# Autodesk Inventor assembly: Bumper Frame
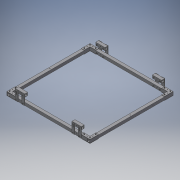
[picture p0: Inventor's stored thumbnail of the model, 180x180]
Saved by Autodesk Inventor 2018 (Build 220112000, 112)
## iProperties
Created: 2019-01-21
Part Number: Bumper Frame
Document SubType Name: Assembly
Designer: maste
Author: maste
## Documents named in this file (8)
- C:\Users\s-2512711\Desktop\Github\2019CAD\Drivebase but Calvin is a mad man\Bumper Frame.iam
- C:\Users\s-2512711\Desktop\Github\2019CAD\Drivebase but Calvin is a mad man\1x1 29in.ipt
- C:\Users\s-2512711\Desktop\Github\2019CAD\Drivebase but Calvin is a mad man\1x1 27in.ipt
- C:\Users\s-2512711\Desktop\Github\2019CAD\Drivebase but Calvin is a mad man\L gusset 2.ipt
- C:\Users\s-2512711\Desktop\Github\2019CAD\Drivebase but Calvin is a mad man\Slot Bumper attachment.ipt
- C:\Users\s-2512711\Desktop\Github\2019CAD\Drivebase but Calvin is a mad man\1x1 Bumper Attachment.ipt
- C:\Users\s-2512711\Desktop\Github\2019CAD\Drivebase but Calvin is a mad man\92196A251_18-8 STAINLESS STEEL SOCKET HEAD CAP SCREW.ipt
- C:\Users\s-2512711\Desktop\Github\2019CAD\Drivebase but Calvin is a mad man\91831A011_TYPE 18-8 STAINLESS STL NYLON-INSERT LOCKNUT.ipt
## Components (80 placed, 7 different names)
1. 1x1 29in:1 — Mate:1, Flush:1, Flush:2, Mate:10, Mate:12, Mate:13, Mate:14, Mate:16, Mate:18, Mate:19, Mate:21
2. 1x1 29in:2 — Mate:2, Flush:3, Flush:4, Mate:3, Flush:5, Flush:6, Mate:4, Mate:5, Mate:7, Mate:9, Mate:24, Mate:26
3. 1x1 27in:1 — Mate:1, Flush:1, Flush:2, Mate:2, Flush:3, Flush:4, Mate:6, Mate:8, Mate:11, Mate:15, Mate:36, Mate:37, Mate:38, Mate:39, Flush:11, Flush:12, Mate:40, Mate:41, Mate:42, Mate:43, Flush:13, Flush:14, Mate:96, Mate:97, Mate:98, Mate:99
4. 1x1 27in:2 — Mate:3, Flush:5, Flush:6, Mate:17, Mate:20, Mate:22, Mate:23, Mate:25, Mate:27, Mate:28, Mate:29, Flush:7, Mate:30, Mate:31, Flush:8, Mate:32, Mate:33, Mate:34, Flush:9, Mate:35, Flush:10, Mate:92, Mate:93, Mate:94, Mate:95
5. L gusset 2:1 — Mate:16, Mate:17, Mate:18, Mate:114, Mate:115, Mate:116
6. L gusset 2:2 — Mate:19, Mate:20, Mate:21, Mate:64, Mate:65, Mate:66, Mate:67, Mate:68, Mate:69
7. L gusset 2:3 — Mate:25, Mate:26, Mate:27, Mate:58, Mate:59, Mate:60, Mate:61, Mate:62, Mate:63
8. L gusset 2:4 — Mate:22, Mate:23, Mate:24, Mate:117, Mate:118, Mate:119
9. L gusset 2:5 — Mate:7, Mate:8, Mate:9, Mate:111, Mate:112, Mate:113
10. L gusset 2:6 — Mate:4, Mate:5, Mate:6, Mate:52, Mate:53, Mate:54, Mate:55, Mate:56, Mate:57
11. L gusset 2:7 — Mate:10, Mate:11, Mate:12, Mate:108, Mate:109, Mate:110
12. L gusset 2:8 — Mate:13, Mate:14, Mate:15, Mate:70, Mate:71, Mate:72, Mate:73, Mate:74, Mate:75
13. Slot Bumper attachment:1 — Mate:32, Mate:35, Flush:10, Mate:44, Mate:45, Flush:15, Mate:87, Mate:91, Mate:149, Mate:150
14. Slot Bumper attachment:2 — Mate:40, Mate:43, Flush:13, Mate:78, Mate:82, Mate:157, Mate:158
15. Slot Bumper attachment:3 — Mate:30, Mate:31, Flush:8, Mate:46, Mate:47, Flush:16, Mate:85, Mate:89, Mate:140, Mate:143
16. Slot Bumper attachment:4 — Mate:28, Mate:29, Flush:7, Mate:84, Mate:88, Mate:141, Mate:142
17. Slot Bumper attachment:5 — Mate:36, Mate:39, Flush:12, Mate:76, Mate:80, Mate:132, Mate:135
18. Slot Bumper attachment:6 — Mate:37, Mate:38, Flush:11, Mate:50, Mate:51, Flush:18, Mate:77, Mate:81, Mate:133, Mate:134
19. Slot Bumper attachment:7 — Mate:33, Mate:34, Flush:9, Mate:86, Mate:90, Mate:148, Mate:151
20. Slot Bumper attachment:8 — Mate:41, Mate:42, Flush:14, Mate:48, Mate:49, Flush:17, Mate:79, Mate:83, Mate:156, Mate:159
21. 1x1 Bumper Attachment:1 — Mate:46, Mate:47, Flush:16, Mate:144, Mate:145
22. 1x1 Bumper Attachment:2 — Mate:50, Mate:51, Flush:18, Mate:136, Mate:137
23. 1x1 Bumper Attachment:3 — Mate:48, Mate:49, Flush:17, Mate:160, Mate:161
24. 1x1 Bumper Attachment:4 — Mate:44, Mate:45, Flush:15, Mate:152, Mate:153
25. 92196A251_18-8 STAINLESS STEEL SOCKET HEAD CAP SCREW:1 — Mate:65, Mate:68, Mate:124
26. 92196A251_18-8 STAINLESS STEEL SOCKET HEAD CAP SCREW:2 — Mate:64, Mate:67, Mate:125
27. 92196A251_18-8 STAINLESS STEEL SOCKET HEAD CAP SCREW:3 — Mate:66, Mate:69, Mate:123
28. 92196A251_18-8 STAINLESS STEEL SOCKET HEAD CAP SCREW:4 — Mate:70, Mate:73, Mate:126
29. 92196A251_18-8 STAINLESS STEEL SOCKET HEAD CAP SCREW:5 — Mate:71, Mate:74, Mate:127
30. 92196A251_18-8 STAINLESS STEEL SOCKET HEAD CAP SCREW:6 — Mate:72, Mate:75, Mate:128
31. 92196A251_18-8 STAINLESS STEEL SOCKET HEAD CAP SCREW:7 — Mate:52, Mate:57, Mate:129
32. 92196A251_18-8 STAINLESS STEEL SOCKET HEAD CAP SCREW:8 — Mate:53, Mate:56, Mate:130
33. 92196A251_18-8 STAINLESS STEEL SOCKET HEAD CAP SCREW:9 — Mate:54, Mate:55, Mate:131
34. 92196A251_18-8 STAINLESS STEEL SOCKET HEAD CAP SCREW:10 — Mate:58, Mate:62, Mate:120
35. 92196A251_18-8 STAINLESS STEEL SOCKET HEAD CAP SCREW:11 — Mate:59, Mate:61, Mate:121
36. 92196A251_18-8 STAINLESS STEEL SOCKET HEAD CAP SCREW:12 — Mate:60, Mate:63, Mate:122
37. 92196A251_18-8 STAINLESS STEEL SOCKET HEAD CAP SCREW:13 — Mate:78, Mate:82, Mate:100
38. 92196A251_18-8 STAINLESS STEEL SOCKET HEAD CAP SCREW:14 — Mate:79, Mate:83, Mate:101
39. 92196A251_18-8 STAINLESS STEEL SOCKET HEAD CAP SCREW:15 — Mate:77, Mate:81, Mate:102
40. 92196A251_18-8 STAINLESS STEEL SOCKET HEAD CAP SCREW:16 — Mate:76, Mate:80, Mate:103
41. 92196A251_18-8 STAINLESS STEEL SOCKET HEAD CAP SCREW:17 — Mate:84, Mate:88, Mate:105
42. 92196A251_18-8 STAINLESS STEEL SOCKET HEAD CAP SCREW:18 — Mate:85, Mate:89, Mate:104
43. 92196A251_18-8 STAINLESS STEEL SOCKET HEAD CAP SCREW:19 — Mate:86, Mate:90, Mate:106
44. 92196A251_18-8 STAINLESS STEEL SOCKET HEAD CAP SCREW:20 — Mate:87, Mate:91, Mate:107
45. 91831A011_TYPE 18-8 STAINLESS STL NYLON-INSERT LOCKNUT:1 — Mate:110, Mate:128
46. 91831A011_TYPE 18-8 STAINLESS STL NYLON-INSERT LOCKNUT:2 — Mate:108, Mate:127
47. 91831A011_TYPE 18-8 STAINLESS STL NYLON-INSERT LOCKNUT:3 — Mate:109, Mate:126
48. 91831A011_TYPE 18-8 STAINLESS STL NYLON-INSERT LOCKNUT:4 — Mate:114, Mate:125
49. 91831A011_TYPE 18-8 STAINLESS STL NYLON-INSERT LOCKNUT:5 — Mate:115, Mate:124
50. 91831A011_TYPE 18-8 STAINLESS STL NYLON-INSERT LOCKNUT:6 — Mate:116, Mate:123
51. 91831A011_TYPE 18-8 STAINLESS STL NYLON-INSERT LOCKNUT:7 — Mate:117, Mate:122
52. 91831A011_TYPE 18-8 STAINLESS STL NYLON-INSERT LOCKNUT:8 — Mate:118, Mate:121
53. 91831A011_TYPE 18-8 STAINLESS STL NYLON-INSERT LOCKNUT:9 — Mate:119, Mate:120
54. 91831A011_TYPE 18-8 STAINLESS STL NYLON-INSERT LOCKNUT:10 — Mate:113, Mate:131
55. 91831A011_TYPE 18-8 STAINLESS STL NYLON-INSERT LOCKNUT:11 — Mate:112, Mate:130
56. 91831A011_TYPE 18-8 STAINLESS STL NYLON-INSERT LOCKNUT:12 — Mate:111, Mate:129
57. 91831A011_TYPE 18-8 STAINLESS STL NYLON-INSERT LOCKNUT:13 — Mate:98, Mate:100
58. 91831A011_TYPE 18-8 STAINLESS STL NYLON-INSERT LOCKNUT:14 — Mate:99, Mate:101
59. 91831A011_TYPE 18-8 STAINLESS STL NYLON-INSERT LOCKNUT:15 — Mate:97, Mate:102
60. 91831A011_TYPE 18-8 STAINLESS STL NYLON-INSERT LOCKNUT:16 — Mate:96, Mate:103
61. 91831A011_TYPE 18-8 STAINLESS STL NYLON-INSERT LOCKNUT:17 — Mate:95, Mate:105
62. 91831A011_TYPE 18-8 STAINLESS STL NYLON-INSERT LOCKNUT:18 — Mate:94, Mate:104
63. 91831A011_TYPE 18-8 STAINLESS STL NYLON-INSERT LOCKNUT:19 — Mate:92, Mate:106
64. 91831A011_TYPE 18-8 STAINLESS STL NYLON-INSERT LOCKNUT:20 — Mate:93, Mate:107
65. 92196A251_18-8 STAINLESS STEEL SOCKET HEAD CAP SCREW:21 — Mate:132, Mate:135, Mate:139
66. 92196A251_18-8 STAINLESS STEEL SOCKET HEAD CAP SCREW:22 — Mate:133, Mate:134, Mate:138
67. 92196A251_18-8 STAINLESS STEEL SOCKET HEAD CAP SCREW:23 — Mate:157, Mate:158, Mate:162
68. 92196A251_18-8 STAINLESS STEEL SOCKET HEAD CAP SCREW:24 — Mate:156, Mate:159, Mate:163
69. 92196A251_18-8 STAINLESS STEEL SOCKET HEAD CAP SCREW:25 — Mate:148, Mate:151, Mate:155
70. 92196A251_18-8 STAINLESS STEEL SOCKET HEAD CAP SCREW:26 — Mate:149, Mate:150, Mate:154
71. 92196A251_18-8 STAINLESS STEEL SOCKET HEAD CAP SCREW:27 — Mate:140, Mate:143, Mate:147
72. 92196A251_18-8 STAINLESS STEEL SOCKET HEAD CAP SCREW:28 — Mate:141, Mate:142, Mate:146
73. 91831A011_TYPE 18-8 STAINLESS STL NYLON-INSERT LOCKNUT:21 — Mate:145, Mate:146
74. 91831A011_TYPE 18-8 STAINLESS STL NYLON-INSERT LOCKNUT:22 — Mate:144, Mate:147
75. 91831A011_TYPE 18-8 STAINLESS STL NYLON-INSERT LOCKNUT:23 — Mate:152, Mate:155
76. 91831A011_TYPE 18-8 STAINLESS STL NYLON-INSERT LOCKNUT:24 — Mate:153, Mate:154
77. 91831A011_TYPE 18-8 STAINLESS STL NYLON-INSERT LOCKNUT:25 — Mate:160, Mate:163
78. 91831A011_TYPE 18-8 STAINLESS STL NYLON-INSERT LOCKNUT:26 — Mate:161, Mate:162
79. 91831A011_TYPE 18-8 STAINLESS STL NYLON-INSERT LOCKNUT:27 — Mate:137, Mate:138
80. 91831A011_TYPE 18-8 STAINLESS STL NYLON-INSERT LOCKNUT:28 — Mate:136, Mate:139
## Relationships (181: Mate 163, Flush 18)
- Mate:1: 1x1 29in:1 ↔ 1x1 27in:1
- Flush:1: 1x1 29in:1 ↔ 1x1 27in:1
- Flush:2: 1x1 29in:1 ↔ 1x1 27in:1
- Mate:2: 1x1 29in:2 ↔ 1x1 27in:1
- Flush:3: 1x1 29in:2 ↔ 1x1 27in:1
- Flush:4: 1x1 29in:2 ↔ 1x1 27in:1
- Mate:3: 1x1 29in:2 ↔ 1x1 27in:2
- Flush:5: 1x1 29in:2 ↔ 1x1 27in:2
- Flush:6: 1x1 29in:2 ↔ 1x1 27in:2
- Mate:4: 1x1 29in:2 ↔ L gusset 2:6
- Mate:5: 1x1 29in:2 ↔ L gusset 2:6
- Mate:6: 1x1 27in:1 ↔ L gusset 2:6
- Mate:7: 1x1 29in:2 ↔ L gusset 2:5
- Mate:8: 1x1 27in:1 ↔ L gusset 2:5
- Mate:9: 1x1 29in:2 ↔ L gusset 2:5
- Mate:10: 1x1 29in:1 ↔ L gusset 2:7
- Mate:11: 1x1 27in:1 ↔ L gusset 2:7
- Mate:12: 1x1 29in:1 ↔ L gusset 2:7
- Mate:13: 1x1 29in:1 ↔ L gusset 2:8
- Mate:14: 1x1 29in:1 ↔ L gusset 2:8
- Mate:15: 1x1 27in:1 ↔ L gusset 2:8
- Mate:16: 1x1 29in:1 ↔ L gusset 2:1
- Mate:17: 1x1 27in:2 ↔ L gusset 2:1
- Mate:18: 1x1 29in:1 ↔ L gusset 2:1
- Mate:19: 1x1 29in:1 ↔ L gusset 2:2
- Mate:20: 1x1 27in:2 ↔ L gusset 2:2
- Mate:21: 1x1 29in:1 ↔ L gusset 2:2
- Mate:22: 1x1 27in:2 ↔ L gusset 2:4
- Mate:23: 1x1 27in:2 ↔ L gusset 2:4
- Mate:24: 1x1 29in:2 ↔ L gusset 2:4
- Mate:25: 1x1 27in:2 ↔ L gusset 2:3
- Mate:26: 1x1 29in:2 ↔ L gusset 2:3
- Mate:27: 1x1 27in:2 ↔ L gusset 2:3
- Mate:28: 1x1 27in:2 ↔ Slot Bumper attachment:4
- Mate:29: 1x1 27in:2 ↔ Slot Bumper attachment:4
- Flush:7: 1x1 27in:2 ↔ Slot Bumper attachment:4
- Mate:30: 1x1 27in:2 ↔ Slot Bumper attachment:3
- Mate:31: 1x1 27in:2 ↔ Slot Bumper attachment:3
- Flush:8: 1x1 27in:2 ↔ Slot Bumper attachment:3
- Mate:32: 1x1 27in:2 ↔ Slot Bumper attachment:1
- Mate:33: 1x1 27in:2 ↔ Slot Bumper attachment:7
- Mate:34: 1x1 27in:2 ↔ Slot Bumper attachment:7
- Flush:9: 1x1 27in:2 ↔ Slot Bumper attachment:7
- Mate:35: 1x1 27in:2 ↔ Slot Bumper attachment:1
- Flush:10: 1x1 27in:2 ↔ Slot Bumper attachment:1
- Mate:36: 1x1 27in:1 ↔ Slot Bumper attachment:5
- Mate:37: 1x1 27in:1 ↔ Slot Bumper attachment:6
- Mate:38: 1x1 27in:1 ↔ Slot Bumper attachment:6
- Mate:39: 1x1 27in:1 ↔ Slot Bumper attachment:5
- Flush:11: 1x1 27in:1 ↔ Slot Bumper attachment:6
- Flush:12: 1x1 27in:1 ↔ Slot Bumper attachment:5
- Mate:40: 1x1 27in:1 ↔ Slot Bumper attachment:2
- Mate:41: 1x1 27in:1 ↔ Slot Bumper attachment:8
- Mate:42: 1x1 27in:1 ↔ Slot Bumper attachment:8
- Mate:43: 1x1 27in:1 ↔ Slot Bumper attachment:2
- Flush:13: 1x1 27in:1 ↔ Slot Bumper attachment:2
- Flush:14: 1x1 27in:1 ↔ Slot Bumper attachment:8
- Mate:44: Slot Bumper attachment:1 ↔ 1x1 Bumper Attachment:4
- Mate:45: Slot Bumper attachment:1 ↔ 1x1 Bumper Attachment:4
- Flush:15: Slot Bumper attachment:1 ↔ 1x1 Bumper Attachment:4
- Mate:46: Slot Bumper attachment:3 ↔ 1x1 Bumper Attachment:1
- Mate:47: Slot Bumper attachment:3 ↔ 1x1 Bumper Attachment:1
- Flush:16: Slot Bumper attachment:3 ↔ 1x1 Bumper Attachment:1
- Mate:48: Slot Bumper attachment:8 ↔ 1x1 Bumper Attachment:3
- Mate:49: Slot Bumper attachment:8 ↔ 1x1 Bumper Attachment:3
- Flush:17: Slot Bumper attachment:8 ↔ 1x1 Bumper Attachment:3
- Mate:50: Slot Bumper attachment:6 ↔ 1x1 Bumper Attachment:2
- Mate:51: Slot Bumper attachment:6 ↔ 1x1 Bumper Attachment:2
- Flush:18: Slot Bumper attachment:6 ↔ 1x1 Bumper Attachment:2
- Mate:52: L gusset 2:6 ↔ 92196A251_18-8 STAINLESS STEEL SOCKET HEAD CAP SCREW:7
- Mate:53: L gusset 2:6 ↔ 92196A251_18-8 STAINLESS STEEL SOCKET HEAD CAP SCREW:8
- Mate:54: L gusset 2:6 ↔ 92196A251_18-8 STAINLESS STEEL SOCKET HEAD CAP SCREW:9
- Mate:55: L gusset 2:6 ↔ 92196A251_18-8 STAINLESS STEEL SOCKET HEAD CAP SCREW:9
- Mate:56: L gusset 2:6 ↔ 92196A251_18-8 STAINLESS STEEL SOCKET HEAD CAP SCREW:8
- Mate:57: L gusset 2:6 ↔ 92196A251_18-8 STAINLESS STEEL SOCKET HEAD CAP SCREW:7
- Mate:58: L gusset 2:3 ↔ 92196A251_18-8 STAINLESS STEEL SOCKET HEAD CAP SCREW:10
- Mate:59: L gusset 2:3 ↔ 92196A251_18-8 STAINLESS STEEL SOCKET HEAD CAP SCREW:11
- Mate:60: L gusset 2:3 ↔ 92196A251_18-8 STAINLESS STEEL SOCKET HEAD CAP SCREW:12
- Mate:61: L gusset 2:3 ↔ 92196A251_18-8 STAINLESS STEEL SOCKET HEAD CAP SCREW:11
- Mate:62: L gusset 2:3 ↔ 92196A251_18-8 STAINLESS STEEL SOCKET HEAD CAP SCREW:10
- Mate:63: L gusset 2:3 ↔ 92196A251_18-8 STAINLESS STEEL SOCKET HEAD CAP SCREW:12
- Mate:64: L gusset 2:2 ↔ 92196A251_18-8 STAINLESS STEEL SOCKET HEAD CAP SCREW:2
- Mate:65: L gusset 2:2 ↔ 92196A251_18-8 STAINLESS STEEL SOCKET HEAD CAP SCREW:1
- Mate:66: L gusset 2:2 ↔ 92196A251_18-8 STAINLESS STEEL SOCKET HEAD CAP SCREW:3
- Mate:67: L gusset 2:2 ↔ 92196A251_18-8 STAINLESS STEEL SOCKET HEAD CAP SCREW:2
- Mate:68: L gusset 2:2 ↔ 92196A251_18-8 STAINLESS STEEL SOCKET HEAD CAP SCREW:1
- Mate:69: L gusset 2:2 ↔ 92196A251_18-8 STAINLESS STEEL SOCKET HEAD CAP SCREW:3
- Mate:70: L gusset 2:8 ↔ 92196A251_18-8 STAINLESS STEEL SOCKET HEAD CAP SCREW:4
- Mate:71: L gusset 2:8 ↔ 92196A251_18-8 STAINLESS STEEL SOCKET HEAD CAP SCREW:5
- Mate:72: L gusset 2:8 ↔ 92196A251_18-8 STAINLESS STEEL SOCKET HEAD CAP SCREW:6
- Mate:73: L gusset 2:8 ↔ 92196A251_18-8 STAINLESS STEEL SOCKET HEAD CAP SCREW:4
- Mate:74: L gusset 2:8 ↔ 92196A251_18-8 STAINLESS STEEL SOCKET HEAD CAP SCREW:5
- Mate:75: L gusset 2:8 ↔ 92196A251_18-8 STAINLESS STEEL SOCKET HEAD CAP SCREW:6
- Mate:76: Slot Bumper attachment:5 ↔ 92196A251_18-8 STAINLESS STEEL SOCKET HEAD CAP SCREW:16
- Mate:77: Slot Bumper attachment:6 ↔ 92196A251_18-8 STAINLESS STEEL SOCKET HEAD CAP SCREW:15
- Mate:78: Slot Bumper attachment:2 ↔ 92196A251_18-8 STAINLESS STEEL SOCKET HEAD CAP SCREW:13
- Mate:79: Slot Bumper attachment:8 ↔ 92196A251_18-8 STAINLESS STEEL SOCKET HEAD CAP SCREW:14
- Mate:80: Slot Bumper attachment:5 ↔ 92196A251_18-8 STAINLESS STEEL SOCKET HEAD CAP SCREW:16
- Mate:81: Slot Bumper attachment:6 ↔ 92196A251_18-8 STAINLESS STEEL SOCKET HEAD CAP SCREW:15
- Mate:82: Slot Bumper attachment:2 ↔ 92196A251_18-8 STAINLESS STEEL SOCKET HEAD CAP SCREW:13
- Mate:83: Slot Bumper attachment:8 ↔ 92196A251_18-8 STAINLESS STEEL SOCKET HEAD CAP SCREW:14
- Mate:84: Slot Bumper attachment:4 ↔ 92196A251_18-8 STAINLESS STEEL SOCKET HEAD CAP SCREW:17
- Mate:85: Slot Bumper attachment:3 ↔ 92196A251_18-8 STAINLESS STEEL SOCKET HEAD CAP SCREW:18
- Mate:86: Slot Bumper attachment:7 ↔ 92196A251_18-8 STAINLESS STEEL SOCKET HEAD CAP SCREW:19
- Mate:87: Slot Bumper attachment:1 ↔ 92196A251_18-8 STAINLESS STEEL SOCKET HEAD CAP SCREW:20
- Mate:88: Slot Bumper attachment:4 ↔ 92196A251_18-8 STAINLESS STEEL SOCKET HEAD CAP SCREW:17
- Mate:89: Slot Bumper attachment:3 ↔ 92196A251_18-8 STAINLESS STEEL SOCKET HEAD CAP SCREW:18
- Mate:90: Slot Bumper attachment:7 ↔ 92196A251_18-8 STAINLESS STEEL SOCKET HEAD CAP SCREW:19
- Mate:91: Slot Bumper attachment:1 ↔ 92196A251_18-8 STAINLESS STEEL SOCKET HEAD CAP SCREW:20
- Mate:92: 1x1 27in:2 ↔ 91831A011_TYPE 18-8 STAINLESS STL NYLON-INSERT LOCKNUT:19
- Mate:93: 1x1 27in:2 ↔ 91831A011_TYPE 18-8 STAINLESS STL NYLON-INSERT LOCKNUT:20
- Mate:94: 1x1 27in:2 ↔ 91831A011_TYPE 18-8 STAINLESS STL NYLON-INSERT LOCKNUT:18
- Mate:95: 1x1 27in:2 ↔ 91831A011_TYPE 18-8 STAINLESS STL NYLON-INSERT LOCKNUT:17
- Mate:96: 1x1 27in:1 ↔ 91831A011_TYPE 18-8 STAINLESS STL NYLON-INSERT LOCKNUT:16
- Mate:97: 1x1 27in:1 ↔ 91831A011_TYPE 18-8 STAINLESS STL NYLON-INSERT LOCKNUT:15
- Mate:98: 1x1 27in:1 ↔ 91831A011_TYPE 18-8 STAINLESS STL NYLON-INSERT LOCKNUT:13
- Mate:99: 1x1 27in:1 ↔ 91831A011_TYPE 18-8 STAINLESS STL NYLON-INSERT LOCKNUT:14
- Mate:100: 92196A251_18-8 STAINLESS STEEL SOCKET HEAD CAP SCREW:13 ↔ 91831A011_TYPE 18-8 STAINLESS STL NYLON-INSERT LOCKNUT:13
- Mate:101: 92196A251_18-8 STAINLESS STEEL SOCKET HEAD CAP SCREW:14 ↔ 91831A011_TYPE 18-8 STAINLESS STL NYLON-INSERT LOCKNUT:14
- Mate:102: 92196A251_18-8 STAINLESS STEEL SOCKET HEAD CAP SCREW:15 ↔ 91831A011_TYPE 18-8 STAINLESS STL NYLON-INSERT LOCKNUT:15
- Mate:103: 92196A251_18-8 STAINLESS STEEL SOCKET HEAD CAP SCREW:16 ↔ 91831A011_TYPE 18-8 STAINLESS STL NYLON-INSERT LOCKNUT:16
- Mate:104: 92196A251_18-8 STAINLESS STEEL SOCKET HEAD CAP SCREW:18 ↔ 91831A011_TYPE 18-8 STAINLESS STL NYLON-INSERT LOCKNUT:18
- Mate:105: 92196A251_18-8 STAINLESS STEEL SOCKET HEAD CAP SCREW:17 ↔ 91831A011_TYPE 18-8 STAINLESS STL NYLON-INSERT LOCKNUT:17
- Mate:106: 92196A251_18-8 STAINLESS STEEL SOCKET HEAD CAP SCREW:19 ↔ 91831A011_TYPE 18-8 STAINLESS STL NYLON-INSERT LOCKNUT:19
- Mate:107: 92196A251_18-8 STAINLESS STEEL SOCKET HEAD CAP SCREW:20 ↔ 91831A011_TYPE 18-8 STAINLESS STL NYLON-INSERT LOCKNUT:20
- Mate:108: L gusset 2:7 ↔ 91831A011_TYPE 18-8 STAINLESS STL NYLON-INSERT LOCKNUT:2
- Mate:109: L gusset 2:7 ↔ 91831A011_TYPE 18-8 STAINLESS STL NYLON-INSERT LOCKNUT:3
- Mate:110: L gusset 2:7 ↔ 91831A011_TYPE 18-8 STAINLESS STL NYLON-INSERT LOCKNUT:1
- Mate:111: L gusset 2:5 ↔ 91831A011_TYPE 18-8 STAINLESS STL NYLON-INSERT LOCKNUT:12
- Mate:112: L gusset 2:5 ↔ 91831A011_TYPE 18-8 STAINLESS STL NYLON-INSERT LOCKNUT:11
- Mate:113: L gusset 2:5 ↔ 91831A011_TYPE 18-8 STAINLESS STL NYLON-INSERT LOCKNUT:10
- Mate:114: L gusset 2:1 ↔ 91831A011_TYPE 18-8 STAINLESS STL NYLON-INSERT LOCKNUT:4
- Mate:115: L gusset 2:1 ↔ 91831A011_TYPE 18-8 STAINLESS STL NYLON-INSERT LOCKNUT:5
- Mate:116: L gusset 2:1 ↔ 91831A011_TYPE 18-8 STAINLESS STL NYLON-INSERT LOCKNUT:6
- Mate:117: L gusset 2:4 ↔ 91831A011_TYPE 18-8 STAINLESS STL NYLON-INSERT LOCKNUT:7
- Mate:118: L gusset 2:4 ↔ 91831A011_TYPE 18-8 STAINLESS STL NYLON-INSERT LOCKNUT:8
- Mate:119: L gusset 2:4 ↔ 91831A011_TYPE 18-8 STAINLESS STL NYLON-INSERT LOCKNUT:9
- Mate:120: 92196A251_18-8 STAINLESS STEEL SOCKET HEAD CAP SCREW:10 ↔ 91831A011_TYPE 18-8 STAINLESS STL NYLON-INSERT LOCKNUT:9
- Mate:121: 92196A251_18-8 STAINLESS STEEL SOCKET HEAD CAP SCREW:11 ↔ 91831A011_TYPE 18-8 STAINLESS STL NYLON-INSERT LOCKNUT:8
- Mate:122: 92196A251_18-8 STAINLESS STEEL SOCKET HEAD CAP SCREW:12 ↔ 91831A011_TYPE 18-8 STAINLESS STL NYLON-INSERT LOCKNUT:7
- Mate:123: 92196A251_18-8 STAINLESS STEEL SOCKET HEAD CAP SCREW:3 ↔ 91831A011_TYPE 18-8 STAINLESS STL NYLON-INSERT LOCKNUT:6
- Mate:124: 92196A251_18-8 STAINLESS STEEL SOCKET HEAD CAP SCREW:1 ↔ 91831A011_TYPE 18-8 STAINLESS STL NYLON-INSERT LOCKNUT:5
- Mate:125: 92196A251_18-8 STAINLESS STEEL SOCKET HEAD CAP SCREW:2 ↔ 91831A011_TYPE 18-8 STAINLESS STL NYLON-INSERT LOCKNUT:4
- Mate:126: 92196A251_18-8 STAINLESS STEEL SOCKET HEAD CAP SCREW:4 ↔ 91831A011_TYPE 18-8 STAINLESS STL NYLON-INSERT LOCKNUT:3
- Mate:127: 92196A251_18-8 STAINLESS STEEL SOCKET HEAD CAP SCREW:5 ↔ 91831A011_TYPE 18-8 STAINLESS STL NYLON-INSERT LOCKNUT:2
- Mate:128: 92196A251_18-8 STAINLESS STEEL SOCKET HEAD CAP SCREW:6 ↔ 91831A011_TYPE 18-8 STAINLESS STL NYLON-INSERT LOCKNUT:1
- Mate:129: 92196A251_18-8 STAINLESS STEEL SOCKET HEAD CAP SCREW:7 ↔ 91831A011_TYPE 18-8 STAINLESS STL NYLON-INSERT LOCKNUT:12
- Mate:130: 92196A251_18-8 STAINLESS STEEL SOCKET HEAD CAP SCREW:8 ↔ 91831A011_TYPE 18-8 STAINLESS STL NYLON-INSERT LOCKNUT:11
- Mate:131: 92196A251_18-8 STAINLESS STEEL SOCKET HEAD CAP SCREW:9 ↔ 91831A011_TYPE 18-8 STAINLESS STL NYLON-INSERT LOCKNUT:10
- Mate:132: Slot Bumper attachment:5 ↔ 92196A251_18-8 STAINLESS STEEL SOCKET HEAD CAP SCREW:21
- Mate:133: Slot Bumper attachment:6 ↔ 92196A251_18-8 STAINLESS STEEL SOCKET HEAD CAP SCREW:22
- Mate:134: Slot Bumper attachment:6 ↔ 92196A251_18-8 STAINLESS STEEL SOCKET HEAD CAP SCREW:22
- Mate:135: Slot Bumper attachment:5 ↔ 92196A251_18-8 STAINLESS STEEL SOCKET HEAD CAP SCREW:21
- Mate:136: 1x1 Bumper Attachment:2 ↔ 91831A011_TYPE 18-8 STAINLESS STL NYLON-INSERT LOCKNUT:28
- Mate:137: 1x1 Bumper Attachment:2 ↔ 91831A011_TYPE 18-8 STAINLESS STL NYLON-INSERT LOCKNUT:27
- Mate:138: 92196A251_18-8 STAINLESS STEEL SOCKET HEAD CAP SCREW:22 ↔ 91831A011_TYPE 18-8 STAINLESS STL NYLON-INSERT LOCKNUT:27
- Mate:139: 92196A251_18-8 STAINLESS STEEL SOCKET HEAD CAP SCREW:21 ↔ 91831A011_TYPE 18-8 STAINLESS STL NYLON-INSERT LOCKNUT:28
- Mate:140: Slot Bumper attachment:3 ↔ 92196A251_18-8 STAINLESS STEEL SOCKET HEAD CAP SCREW:27
- Mate:141: Slot Bumper attachment:4 ↔ 92196A251_18-8 STAINLESS STEEL SOCKET HEAD CAP SCREW:28
- Mate:142: Slot Bumper attachment:4 ↔ 92196A251_18-8 STAINLESS STEEL SOCKET HEAD CAP SCREW:28
- Mate:143: Slot Bumper attachment:3 ↔ 92196A251_18-8 STAINLESS STEEL SOCKET HEAD CAP SCREW:27
- Mate:144: 1x1 Bumper Attachment:1 ↔ 91831A011_TYPE 18-8 STAINLESS STL NYLON-INSERT LOCKNUT:22
- Mate:145: 1x1 Bumper Attachment:1 ↔ 91831A011_TYPE 18-8 STAINLESS STL NYLON-INSERT LOCKNUT:21
- Mate:146: 92196A251_18-8 STAINLESS STEEL SOCKET HEAD CAP SCREW:28 ↔ 91831A011_TYPE 18-8 STAINLESS STL NYLON-INSERT LOCKNUT:21
- Mate:147: 92196A251_18-8 STAINLESS STEEL SOCKET HEAD CAP SCREW:27 ↔ 91831A011_TYPE 18-8 STAINLESS STL NYLON-INSERT LOCKNUT:22
- Mate:148: Slot Bumper attachment:7 ↔ 92196A251_18-8 STAINLESS STEEL SOCKET HEAD CAP SCREW:25
- Mate:149: Slot Bumper attachment:1 ↔ 92196A251_18-8 STAINLESS STEEL SOCKET HEAD CAP SCREW:26
- Mate:150: Slot Bumper attachment:1 ↔ 92196A251_18-8 STAINLESS STEEL SOCKET HEAD CAP SCREW:26
- Mate:151: Slot Bumper attachment:7 ↔ 92196A251_18-8 STAINLESS STEEL SOCKET HEAD CAP SCREW:25
- Mate:152: 1x1 Bumper Attachment:4 ↔ 91831A011_TYPE 18-8 STAINLESS STL NYLON-INSERT LOCKNUT:23
- Mate:153: 1x1 Bumper Attachment:4 ↔ 91831A011_TYPE 18-8 STAINLESS STL NYLON-INSERT LOCKNUT:24
- Mate:154: 92196A251_18-8 STAINLESS STEEL SOCKET HEAD CAP SCREW:26 ↔ 91831A011_TYPE 18-8 STAINLESS STL NYLON-INSERT LOCKNUT:24
- Mate:155: 92196A251_18-8 STAINLESS STEEL SOCKET HEAD CAP SCREW:25 ↔ 91831A011_TYPE 18-8 STAINLESS STL NYLON-INSERT LOCKNUT:23
- Mate:156: Slot Bumper attachment:8 ↔ 92196A251_18-8 STAINLESS STEEL SOCKET HEAD CAP SCREW:24
- Mate:157: Slot Bumper attachment:2 ↔ 92196A251_18-8 STAINLESS STEEL SOCKET HEAD CAP SCREW:23
- Mate:158: Slot Bumper attachment:2 ↔ 92196A251_18-8 STAINLESS STEEL SOCKET HEAD CAP SCREW:23
- Mate:159: Slot Bumper attachment:8 ↔ 92196A251_18-8 STAINLESS STEEL SOCKET HEAD CAP SCREW:24
- Mate:160: 1x1 Bumper Attachment:3 ↔ 91831A011_TYPE 18-8 STAINLESS STL NYLON-INSERT LOCKNUT:25
- Mate:161: 1x1 Bumper Attachment:3 ↔ 91831A011_TYPE 18-8 STAINLESS STL NYLON-INSERT LOCKNUT:26
- Mate:162: 92196A251_18-8 STAINLESS STEEL SOCKET HEAD CAP SCREW:23 ↔ 91831A011_TYPE 18-8 STAINLESS STL NYLON-INSERT LOCKNUT:26
- Mate:163: 92196A251_18-8 STAINLESS STEEL SOCKET HEAD CAP SCREW:24 ↔ 91831A011_TYPE 18-8 STAINLESS STL NYLON-INSERT LOCKNUT:25
